# Autodesk Inventor assembly: Assembly1
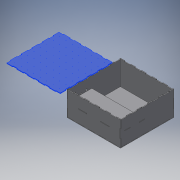
[picture p0: Inventor's stored thumbnail of the model, 180x180]
Saved by Autodesk Inventor 2016 (Build 200138000, 138)
## iProperties
Created: 2016-12-12
Part Number: Assembly1
Document SubType Name: Assembly
Designer: NacostaMobile
Author: NacostaMobile
## Documents named in this file (8)
- D:\Nacosta\Documents\UC\La resistencia\Cubo\Assembly1.iam
- D:\Nacosta\Documents\UC\La resistencia\Cubo\Btapa.ipt
- D:\Nacosta\Documents\UC\La resistencia\Cubo\latGenerico.ipt
- D:\Nacosta\Documents\UC\La resistencia\Cubo\latBack.ipt
- D:\Nacosta\Documents\UC\La resistencia\Cubo\latPort.ipt
- D:\Nacosta\Documents\UC\La resistencia\Cubo\latOpSupp.ipt
- D:\Nacosta\Documents\UC\La resistencia\Cubo\InSupp.ipt
- D:\Nacosta\Documents\UC\La resistencia\Cubo\BtapaHole.ipt
## Components (7 placed, 7 different names)
1. Btapa:1 — Mate:1, Mate:2, Mate:3, Mate:5, Mate:6
2. latBack:1 — Mate:5, Mate:10
3. latPort:1 — Mate:3, Mate:4, Mate:9
4. latOpSupp:1 — Mate:6, Mate:7, Mate:8
5. InSupp:1 — Mate:7, Mate:8, Mate:9, Mate:10
6. latGenerico:1 — Mate:1, Mate:2, Mate:4
7. BtapaHole:1
## Relationships (10: Mate 10)
- Mate:1: Btapa:1 ↔ latGenerico:1
- Mate:2: Btapa:1 ↔ latGenerico:1
- Mate:3: Btapa:1 ↔ latPort:1
- Mate:4: latPort:1 ↔ latGenerico:1
- Mate:5: Btapa:1 ↔ latBack:1
- Mate:6: Btapa:1 ↔ latOpSupp:1
- Mate:7: latOpSupp:1 ↔ InSupp:1
- Mate:8: latOpSupp:1 ↔ InSupp:1
- Mate:9: latPort:1 ↔ InSupp:1
- Mate:10: latBack:1 ↔ InSupp:1
